# Autodesk Inventor assembly: BungaSign-Biggerv2
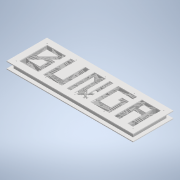
[picture p0: Inventor's stored thumbnail of the model, 180x180]
Saved by Autodesk Inventor 2022 (Build 260153000, 153)
## iProperties
Created: 2022-08-17
Part Number: BungaSign-Biggerv2
Document SubType Name: Assembly
Designer: incep
Author: incep
## Documents named in this file (10)
- C:\Users\incep\OneDrive\Desktop\Laser Cutter Things\BungaSign-Biggerv2.iam
- C:\Users\incep\OneDrive\Desktop\Laser Cutter Things\BungaSign-Bigger.ipt
- C:\Users\incep\OneDrive\Desktop\Laser Cutter Things\BungaSign-Bigger-Layer1v2.ipt
- C:\Users\incep\OneDrive\Desktop\Laser Cutter Things\BungaSign-Bigger-Layer2v2.ipt
- C:\Users\incep\OneDrive\Desktop\Laser Cutter Things\BungaSign-Bigger-Layer3v2.ipt
- C:\Users\incep\OneDrive\Desktop\Laser Cutter Things\BungaSign-Bigger-Layer4v2.ipt
- C:\Users\incep\OneDrive\Desktop\Laser Cutter Things\BungaSign-Bigger-Layer5v2.ipt
- C:\Users\incep\OneDrive\Desktop\Laser Cutter Things\BungaSign-Bigger-Layer6v2.ipt
- C:\Users\incep\OneDrive\Desktop\Laser Cutter Things\BungaSign-Bigger-Layer7v2.ipt
- C:\Users\incep\OneDrive\Desktop\Laser Cutter Things\BungaSign-Bigger-Back.ipt
## Components (9 placed, 9 different names)
1. BungaSign-Bigger:1 — Flush:1, Mate:1, Mate:2, Mate:3, Mate:6, Mate:8, Mate:9, Mate:12, Mate:15, Mate:17, Mate:18, Mate:20, Mate:21, Mate:23, Mate:24
2. BungaSign-Bigger-Layer1v2:1 — Mate:1, Mate:2, Mate:3, Mate:4, Mate:5
3. BungaSign-Bigger-Layer2v2:1 — Mate:4, Mate:5, Mate:6, Mate:7
4. BungaSign-Bigger-Layer3v2:1 — Mate:7, Mate:8, Mate:9, Mate:10, Mate:11
5. BungaSign-Bigger-Layer4v2:1 — Mate:10, Mate:11, Mate:12, Mate:13, Mate:14
6. BungaSign-Bigger-Layer5v2:1 — Mate:13, Mate:14, Mate:15, Mate:16
7. BungaSign-Bigger-Layer6v2:1 — Mate:16, Mate:17, Mate:18, Mate:19
8. BungaSign-Bigger-Layer7v2:1 — Mate:19, Mate:20, Mate:21, Mate:22
9. BungaSign-Bigger-Back:1 — Mate:22, Mate:23, Mate:24
## Relationships (25: Mate 24, Flush 1)
- Flush:1: BungaSign-Bigger:1
- Mate:1: BungaSign-Bigger:1 ↔ BungaSign-Bigger-Layer1v2:1
- Mate:2: BungaSign-Bigger:1 ↔ BungaSign-Bigger-Layer1v2:1
- Mate:3: BungaSign-Bigger:1 ↔ BungaSign-Bigger-Layer1v2:1
- Mate:4: BungaSign-Bigger-Layer1v2:1 ↔ BungaSign-Bigger-Layer2v2:1
- Mate:5: BungaSign-Bigger-Layer1v2:1 ↔ BungaSign-Bigger-Layer2v2:1
- Mate:6: BungaSign-Bigger:1 ↔ BungaSign-Bigger-Layer2v2:1
- Mate:7: BungaSign-Bigger-Layer2v2:1 ↔ BungaSign-Bigger-Layer3v2:1
- Mate:8: BungaSign-Bigger:1 ↔ BungaSign-Bigger-Layer3v2:1
- Mate:9: BungaSign-Bigger:1 ↔ BungaSign-Bigger-Layer3v2:1
- Mate:10: BungaSign-Bigger-Layer3v2:1 ↔ BungaSign-Bigger-Layer4v2:1
- Mate:11: BungaSign-Bigger-Layer3v2:1 ↔ BungaSign-Bigger-Layer4v2:1
- Mate:12: BungaSign-Bigger:1 ↔ BungaSign-Bigger-Layer4v2:1
- Mate:13: BungaSign-Bigger-Layer4v2:1 ↔ BungaSign-Bigger-Layer5v2:1
- Mate:14: BungaSign-Bigger-Layer4v2:1 ↔ BungaSign-Bigger-Layer5v2:1
- Mate:15: BungaSign-Bigger:1 ↔ BungaSign-Bigger-Layer5v2:1
- Mate:16: BungaSign-Bigger-Layer5v2:1 ↔ BungaSign-Bigger-Layer6v2:1
- Mate:17: BungaSign-Bigger:1 ↔ BungaSign-Bigger-Layer6v2:1
- Mate:18: BungaSign-Bigger:1 ↔ BungaSign-Bigger-Layer6v2:1
- Mate:19: BungaSign-Bigger-Layer6v2:1 ↔ BungaSign-Bigger-Layer7v2:1
- Mate:20: BungaSign-Bigger:1 ↔ BungaSign-Bigger-Layer7v2:1
- Mate:21: BungaSign-Bigger:1 ↔ BungaSign-Bigger-Layer7v2:1
- Mate:22: BungaSign-Bigger-Layer7v2:1 ↔ BungaSign-Bigger-Back:1
- Mate:23: BungaSign-Bigger:1 ↔ BungaSign-Bigger-Back:1
- Mate:24: BungaSign-Bigger:1 ↔ BungaSign-Bigger-Back:1
